# Autodesk Inventor assembly: Beslag_til_stempel'
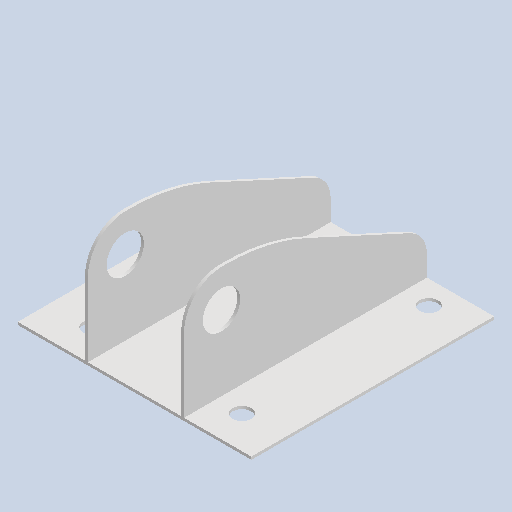
[picture p0: Inventor's stored thumbnail of the model, 512x512]
Saved by Autodesk Inventor 2022 (Build 260153000, 153)
## iProperties
Created: 2022-04-09
Part Number: Beslag_til_stempel'
Document SubType Name: Assembly
Designer: Patrick
Author: Patrick
## Documents named in this file (3)
- H:\OneDrive - Syddansk Universitet\2. Semester Master\Mekaniske Elementer\Mini Project\2020-10-23\Workspaces\Workspace\Beslag_til_stempel'.iam
- H:\OneDrive - Syddansk Universitet\2. Semester Master\Mekaniske Elementer\Mini Project\2020-10-23\Workspaces\Workspace\Beslag_stempel.ipt
- H:\OneDrive - Syddansk Universitet\2. Semester Master\Mekaniske Elementer\Mini Project\2020-10-23\Workspaces\Workspace\plade_til_beslag.ipt
## Components (3 placed, 2 different names)
1. Beslag_stempel:1 — Mate:1, Flush:1, Flush:2
2. Beslag_stempel:2 — Flush:3, Flush:4, Mate:2
3. plade_til_beslag:1 — Mate:1, Flush:1, Flush:2, Flush:3, Flush:4, Mate:2
## Relationships (6: Flush 4, Mate 2)
- Mate:1: Beslag_stempel:1 ↔ plade_til_beslag:1
- Flush:1: Beslag_stempel:1 ↔ plade_til_beslag:1
- Flush:2 (36 mm): Beslag_stempel:1 ↔ plade_til_beslag:1
- Flush:3 (36 mm): Beslag_stempel:2 ↔ plade_til_beslag:1
- Flush:4: Beslag_stempel:2 ↔ plade_til_beslag:1
- Mate:2: Beslag_stempel:2 ↔ plade_til_beslag:1
